# Autodesk Inventor assembly: robot
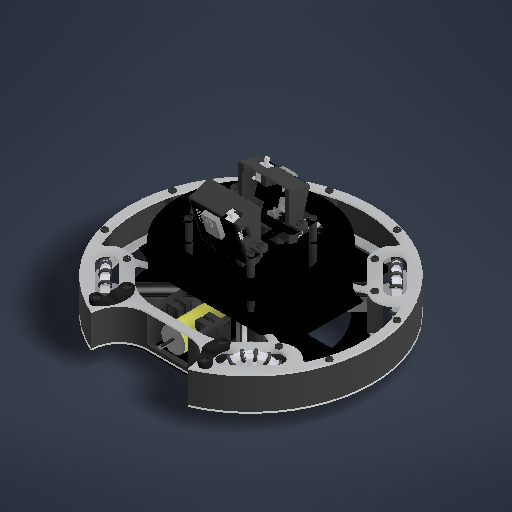
[picture p0: Inventor's stored thumbnail of the model, 512x512]
Saved by Autodesk Inventor 2025.2 (Build 292293000, 293)
## iProperties
Created: 2023-05-12
Part Number: robot
Document SubType Name: Assembly
Designer: Elias Braun
Author: Elias Braun
## Documents named in this file (7)
- C:\Users\EliasBraun\Nextcloud2\RoboCup2023 - WM\robot.iam
- C:\Users\EliasBraun\Nextcloud2\RoboCup2023 - WM\Substructure.iam
- C:\Users\EliasBraun\Nextcloud2\RoboCup2023 - WM\Suberstructure.iam
- C:\Users\EliasBraun\Nextcloud2\RoboCup2023 - WM\Connectors\Controller-IR-Spacer(FusionThread).ipt
- C:\Users\EliasBraun\Nextcloud2\RoboCup2023 - WM\Miscellaneous\LightBarrier-Brackets.ipt
- C:\Users\EliasBraun\Nextcloud2\RoboCup2023 - WM\Fasteners\ISO 7380-1 - M3 x 30.ipt
- C:\Users\EliasBraun\Nextcloud2\RoboCup2023 - WM\Fasteners\ISO 7380-1 - M3 x 8.ipt
## Components (31 placed, 6 different names)
1. Substructure:1 [sub-assembly] — Mate:1, Mate:2, Mate:3, Mate:4, Mate:5, Mate:6, Mate:7, Mate:8, Mate:12, Mate:13, Mate:14, Mate:17, Mate:18, Mate:19, Mate:20, Mate:21, Mate:22, Mate:23, Mate:24, Mate:25, Mate:26, Mate:27, Mate:28, Mate:32, Mate:34, Mate:35, Mate:36, Mate:37, Mate:38, Mate:55, Mate:57, Mate:58, Mate:59, Mate:60, Mate:62
2. Suberstructure:1 [sub-assembly] — Mate:9, Mate:10, Mate:11, Mate:39, Mate:40, Mate:41, Mate:42, Mate:43, Mate:44, Mate:45, Mate:46, Mate:47, Mate:48, Mate:49, Mate:50, Mate:51, Mate:52, Mate:53, Mate:54
3. Controller-IR-Spacer(FusionThread):1 — Mate:1, Mate:6
4. Controller-IR-Spacer(FusionThread):2 — Mate:3, Mate:8, Mate:9, Mate:11
5. Controller-IR-Spacer(FusionThread):3 — Mate:4, Mate:7, Mate:10
6. Controller-IR-Spacer(FusionThread):4 — Mate:2, Mate:5
7. LightBarrier-Brackets:1 — Mate:12, Mate:13, Mate:14, Mate:15, Mate:16, Mate:29, Mate:30, Mate:31, Mate:33, Mate:56, Mate:61
8. ISO 7380-1 M3 x 30:1 — Mate:15, Mate:30
9. ISO 7380-1 M3 x 30:2 — Mate:21, Mate:23
10. ISO 7380-1 M3 x 30:3 — Mate:22, Mate:24
11. ISO 7380-1 M3 x 30:4 — Mate:18, Mate:27
12. ISO 7380-1 M3 x 30:5 — Mate:17, Mate:28
13. ISO 7380-1 M3 x 30:6 — Mate:16, Mate:29
14. ISO 7380-1 M3 x 30:7 — Mate:20, Mate:25
15. ISO 7380-1 M3 x 30:8 — Mate:19, Mate:26
16. ISO 7380-1 M3 x 8:1 — Mate:31, Mate:61
17. ISO 7380-1 M3 x 8:2 — Mate:32, Mate:62
18. ISO 7380-1 M3 x 8:3 — Mate:33, Mate:56
19. ISO 7380-1 M3 x 8:4 — Mate:34, Mate:55
20. ISO 7380-1 M3 x 8:5 — Mate:35, Mate:57
21. ISO 7380-1 M3 x 8:6 — Mate:36, Mate:58
22. ISO 7380-1 M3 x 8:7 — Mate:37, Mate:59
23. ISO 7380-1 M3 x 8:8 — Mate:38, Mate:60
24. ISO 7380-1 M3 x 8:9 — Mate:46, Mate:49
25. ISO 7380-1 M3 x 8:10 — Mate:44, Mate:48
26. ISO 7380-1 M3 x 8:11 — Mate:43, Mate:53
27. ISO 7380-1 M3 x 8:12 — Mate:45, Mate:52
28. ISO 7380-1 M3 x 8:13 — Mate:40, Mate:47
29. ISO 7380-1 M3 x 8:14 — Mate:42, Mate:50
30. ISO 7380-1 M3 x 8:15 — Mate:41, Mate:51
31. ISO 7380-1 M3 x 8:16 — Mate:39, Mate:54
## Relationships (62: Mate 62)
- Mate:1: Substructure:1 ↔ Controller-IR-Spacer(FusionThread):1
- Mate:2: Substructure:1 ↔ Controller-IR-Spacer(FusionThread):4
- Mate:3: Substructure:1 ↔ Controller-IR-Spacer(FusionThread):2
- Mate:4: Substructure:1 ↔ Controller-IR-Spacer(FusionThread):3
- Mate:5: Substructure:1 ↔ Controller-IR-Spacer(FusionThread):4
- Mate:6: Substructure:1 ↔ Controller-IR-Spacer(FusionThread):1
- Mate:7: Substructure:1 ↔ Controller-IR-Spacer(FusionThread):3
- Mate:8: Substructure:1 ↔ Controller-IR-Spacer(FusionThread):2
- Mate:9: Suberstructure:1 ↔ Controller-IR-Spacer(FusionThread):2
- Mate:10: Suberstructure:1 ↔ Controller-IR-Spacer(FusionThread):3
- Mate:11: Suberstructure:1 ↔ Controller-IR-Spacer(FusionThread):2
- Mate:12: Substructure:1 ↔ LightBarrier-Brackets:1
- Mate:13: Substructure:1 ↔ LightBarrier-Brackets:1
- Mate:14: Substructure:1 ↔ LightBarrier-Brackets:1
- Mate:15: LightBarrier-Brackets:1 ↔ ISO 7380-1 M3 x 30:1
- Mate:16: LightBarrier-Brackets:1 ↔ ISO 7380-1 M3 x 30:6
- Mate:17: Substructure:1 ↔ ISO 7380-1 M3 x 30:5
- Mate:18: Substructure:1 ↔ ISO 7380-1 M3 x 30:4
- Mate:19: Substructure:1 ↔ ISO 7380-1 M3 x 30:8
- Mate:20: Substructure:1 ↔ ISO 7380-1 M3 x 30:7
- Mate:21: Substructure:1 ↔ ISO 7380-1 M3 x 30:2
- Mate:22: Substructure:1 ↔ ISO 7380-1 M3 x 30:3
- Mate:23: Substructure:1 ↔ ISO 7380-1 M3 x 30:2
- Mate:24: Substructure:1 ↔ ISO 7380-1 M3 x 30:3
- Mate:25: Substructure:1 ↔ ISO 7380-1 M3 x 30:7
- Mate:26: Substructure:1 ↔ ISO 7380-1 M3 x 30:8
- Mate:27: Substructure:1 ↔ ISO 7380-1 M3 x 30:4
- Mate:28: Substructure:1 ↔ ISO 7380-1 M3 x 30:5
- Mate:29: LightBarrier-Brackets:1 ↔ ISO 7380-1 M3 x 30:6
- Mate:30: LightBarrier-Brackets:1 ↔ ISO 7380-1 M3 x 30:1
- Mate:31: LightBarrier-Brackets:1 ↔ ISO 7380-1 M3 x 8:1
- Mate:32: Substructure:1 ↔ ISO 7380-1 M3 x 8:2
- Mate:33: LightBarrier-Brackets:1 ↔ ISO 7380-1 M3 x 8:3
- Mate:34: Substructure:1 ↔ ISO 7380-1 M3 x 8:4
- Mate:35: Substructure:1 ↔ ISO 7380-1 M3 x 8:5
- Mate:36: Substructure:1 ↔ ISO 7380-1 M3 x 8:6
- Mate:37: Substructure:1 ↔ ISO 7380-1 M3 x 8:7
- Mate:38: Substructure:1 ↔ ISO 7380-1 M3 x 8:8
- Mate:39: Suberstructure:1 ↔ ISO 7380-1 M3 x 8:16
- Mate:40: Suberstructure:1 ↔ ISO 7380-1 M3 x 8:13
- Mate:41: Suberstructure:1 ↔ ISO 7380-1 M3 x 8:15
- Mate:42: Suberstructure:1 ↔ ISO 7380-1 M3 x 8:14
- Mate:43: Suberstructure:1 ↔ ISO 7380-1 M3 x 8:11
- Mate:44: Suberstructure:1 ↔ ISO 7380-1 M3 x 8:10
- Mate:45: Suberstructure:1 ↔ ISO 7380-1 M3 x 8:12
- Mate:46: Suberstructure:1 ↔ ISO 7380-1 M3 x 8:9
- Mate:47: Suberstructure:1 ↔ ISO 7380-1 M3 x 8:13
- Mate:48: Suberstructure:1 ↔ ISO 7380-1 M3 x 8:10
- Mate:49: Suberstructure:1 ↔ ISO 7380-1 M3 x 8:9
- Mate:50: Suberstructure:1 ↔ ISO 7380-1 M3 x 8:14
- Mate:51: Suberstructure:1 ↔ ISO 7380-1 M3 x 8:15
- Mate:52: Suberstructure:1 ↔ ISO 7380-1 M3 x 8:12
- Mate:53: Suberstructure:1 ↔ ISO 7380-1 M3 x 8:11
- Mate:54: Suberstructure:1 ↔ ISO 7380-1 M3 x 8:16
- Mate:55: Substructure:1 ↔ ISO 7380-1 M3 x 8:4
- Mate:56: LightBarrier-Brackets:1 ↔ ISO 7380-1 M3 x 8:3
- Mate:57: Substructure:1 ↔ ISO 7380-1 M3 x 8:5
- Mate:58: Substructure:1 ↔ ISO 7380-1 M3 x 8:6
- Mate:59: Substructure:1 ↔ ISO 7380-1 M3 x 8:7
- Mate:60: Substructure:1 ↔ ISO 7380-1 M3 x 8:8
- Mate:61: LightBarrier-Brackets:1 ↔ ISO 7380-1 M3 x 8:1
- Mate:62: Substructure:1 ↔ ISO 7380-1 M3 x 8:2
